# Autodesk Inventor assembly: A2017_T4_06
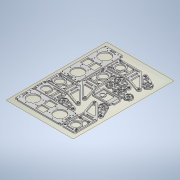
[picture p0: Inventor's stored thumbnail of the model, 180x180]
Saved by Autodesk Inventor 2020 (Build 240168000, 168)
## iProperties
Created: 2021-08-27
Part Number: A2017_T4_06
Document SubType Name: Assembly
Designer: Masato
Author: Masato
## Documents named in this file (10)
- C:\Users\naoki\Documents\Inventor\CitBrains\git_clone\SUSTAINA_ver1_0\AT5_175\SUSTAINA-OP\Cam\A2017_T4_06.iam
- C:\Users\naoki\Documents\Inventor\CitBrains\git_clone\SUSTAINA_ver1_0\AT5_175\SUSTAINA-OP\Cam\DisposableBoard.ipt
- C:\Users\naoki\Documents\Inventor\CitBrains\git_clone\SUSTAINA_ver1_0\AT5_175\SUSTAINA-OP\LowerBody\Ankle\Ankle_side_pitch_frame.ipt
- C:\Users\naoki\Documents\Inventor\CitBrains\git_clone\SUSTAINA_ver1_0\AT5_175\SUSTAINA-OP\UpperBody\Trunk\Trunk_neck_frame.ipt
- C:\Users\naoki\Documents\Inventor\CitBrains\git_clone\SUSTAINA_ver1_0\AT5_175\SUSTAINA-OP\UpperBody\Trunk\Trunk_shoulder_frame.ipt
- C:\Users\naoki\Documents\Inventor\CitBrains\git_clone\SUSTAINA_ver1_0\AT5_175\SUSTAINA-OP\UpperBody\Trunk\Trunk_shoulder_frame_MIR.ipt
- C:\Users\naoki\Documents\Inventor\CitBrains\git_clone\SUSTAINA_ver1_0\AT5_175\SUSTAINA-OP\UpperBody\Trunk\Trunk_waisit_frame.ipt
- C:\Users\naoki\Documents\Inventor\CitBrains\git_clone\SUSTAINA_ver1_0\AT5_175\SUSTAINA-OP\UpperBody\Trunk\Trunk_servo_bottom_frame.ipt
- C:\Users\naoki\Documents\Inventor\CitBrains\git_clone\SUSTAINA_ver1_0\AT4_173\SUSTAINA-OP\UpperBody\Trunk\Trunk_shoulder_frame.ipt
- C:\Users\naoki\Documents\Inventor\CitBrains\git_clone\SUSTAINA_ver1_0\AT4_173\SUSTAINA-OP\UpperBody\Trunk\Trunk_shoulder_frame_MIR.ipt
## Components (15 placed, 7 different names)
1. DisposableBoard:1 — メイト:2, メイト:1, フラッシュ:1, フラッシュ:2, フラッシュ:3, フラッシュ:5, メイト:27, メイト:28, メイト:29, メイト:37, メイト:38, フラッシュ:8, メイト:43, メイト:44, 角度:1, 正接:6, 正接:9
2. Trunk_neck_frame:1 — メイト:6, フラッシュ:6, フラッシュ:7, メイト:16, メイト:17, 正接:2
3. Trunk_shoulder_frame:1 — メイト:9, フラッシュ:4, メイト:15, メイト:45, 正接:3
4. Trunk_shoulder_frame_MIR:1 — メイト:10, フラッシュ:7, メイト:17, メイト:42, メイト:46
5. Trunk_waisit_frame:1 — フラッシュ:3, フラッシュ:4, フラッシュ:5, フラッシュ:6, メイト:15, メイト:16, メイト:19
6. Ankle_side_pitch_frame:2 — メイト:5, メイト:19, 正接:2
7. Ankle_side_pitch_frame:1 — メイト:4, メイト:45, 正接:3, 正接:4
8. Trunk_servo_bottom_frame:2 — メイト:14, 正接:4, メイト:48, 角度:1, メイト:49
9. Trunk_waisit_frame:2 — メイト:27, メイト:42, フラッシュ:8, メイト:47, メイト:52
10. Ankle_side_pitch_frame:6 — メイト:29, メイト:53, 正接:9
11. Ankle_side_pitch_frame:7 — メイト:28, メイト:51, 正接:7, 正接:8
12. Ankle_side_pitch_frame:8 — メイト:37, メイト:50, 正接:5, メイト:51
13. Ankle_side_pitch_frame:9 — メイト:38, メイト:49, メイト:50, 正接:6
14. Trunk_shoulder_frame:2 — メイト:44, メイト:46, メイト:47, メイト:48, 正接:5, 正接:7
15. Trunk_shoulder_frame_MIR:2 — メイト:43, 正接:8, メイト:52, メイト:53
## Relationships (46: Mate 29, Flush 8, Tangent 8, Angle 1)
- メイト:2 [Mate]: DisposableBoard:1
- メイト:1 [Mate]: DisposableBoard:1
- フラッシュ:1 [Flush]: DisposableBoard:1
- フラッシュ:2 [Flush]: DisposableBoard:1
- メイト:4 [Mate]: Ankle_side_pitch_frame:1
- メイト:5 [Mate]: Ankle_side_pitch_frame:2
- メイト:6 [Mate]: Trunk_neck_frame:1
- メイト:9 [Mate]: Trunk_shoulder_frame:1
- メイト:10 [Mate]: Trunk_shoulder_frame_MIR:1
- メイト:14 [Mate]: Trunk_servo_bottom_frame:2
- フラッシュ:3 [Flush] (2 mm): DisposableBoard:1 ↔ Trunk_waisit_frame:1
- フラッシュ:4 [Flush]: Trunk_shoulder_frame:1 ↔ Trunk_waisit_frame:1
- フラッシュ:5 [Flush] (2 mm): DisposableBoard:1 ↔ Trunk_waisit_frame:1
- フラッシュ:6 [Flush]: Trunk_neck_frame:1 ↔ Trunk_waisit_frame:1
- フラッシュ:7 [Flush]: Trunk_neck_frame:1 ↔ Trunk_shoulder_frame_MIR:1
- メイト:15 [Mate] (2.5 mm): Trunk_shoulder_frame:1 ↔ Trunk_waisit_frame:1
- メイト:16 [Mate] (2.5 mm): Trunk_neck_frame:1 ↔ Trunk_waisit_frame:1
- メイト:17 [Mate] (2.5 mm): Trunk_neck_frame:1 ↔ Trunk_shoulder_frame_MIR:1
- メイト:19 [Mate] (2.5 mm): Trunk_waisit_frame:1 ↔ Ankle_side_pitch_frame:2
- 正接:2 [Tangent] (2.5 mm): Trunk_neck_frame:1 ↔ Ankle_side_pitch_frame:2
- メイト:27 [Mate]: DisposableBoard:1 ↔ Trunk_waisit_frame:2
- メイト:28 [Mate]: DisposableBoard:1 ↔ Ankle_side_pitch_frame:7
- メイト:29 [Mate]: DisposableBoard:1 ↔ Ankle_side_pitch_frame:6
- メイト:37 [Mate]: DisposableBoard:1 ↔ Ankle_side_pitch_frame:8
- メイト:38 [Mate]: DisposableBoard:1 ↔ Ankle_side_pitch_frame:9
- メイト:42 [Mate] (2.5 mm): Trunk_shoulder_frame_MIR:1 ↔ Trunk_waisit_frame:2
- フラッシュ:8 [Flush] (2.5 mm): DisposableBoard:1 ↔ Trunk_waisit_frame:2
- メイト:43 [Mate]: DisposableBoard:1 ↔ Trunk_shoulder_frame_MIR:2
- メイト:44 [Mate]: DisposableBoard:1 ↔ Trunk_shoulder_frame:2
- メイト:45 [Mate] (2.5 mm): Trunk_shoulder_frame:1 ↔ Ankle_side_pitch_frame:1
- 正接:3 [Tangent]: Trunk_shoulder_frame:1 ↔ Ankle_side_pitch_frame:1
- メイト:46 [Mate] (2.5 mm): Trunk_shoulder_frame_MIR:1 ↔ Trunk_shoulder_frame:2
- メイト:47 [Mate] (2.5 mm): Trunk_waisit_frame:2 ↔ Trunk_shoulder_frame:2
- 正接:4 [Tangent] (2.5 mm): Ankle_side_pitch_frame:1 ↔ Trunk_servo_bottom_frame:2
- メイト:48 [Mate] (2.5 mm): Trunk_servo_bottom_frame:2 ↔ Trunk_shoulder_frame:2
- 角度:1 [Angle] (0 deg): DisposableBoard:1 ↔ Trunk_servo_bottom_frame:2
- メイト:49 [Mate] (2.5 mm): Trunk_servo_bottom_frame:2 ↔ Ankle_side_pitch_frame:9
- メイト:50 [Mate] (2.5 mm): Ankle_side_pitch_frame:8 ↔ Ankle_side_pitch_frame:9
- 正接:5 [Tangent] (2.5 mm): Ankle_side_pitch_frame:8 ↔ Trunk_shoulder_frame:2
- 正接:6 [Tangent] (3 mm): DisposableBoard:1 ↔ Ankle_side_pitch_frame:9
- メイト:51 [Mate] (2.5 mm): Ankle_side_pitch_frame:7 ↔ Ankle_side_pitch_frame:8
- 正接:7 [Tangent] (2.5 mm): Ankle_side_pitch_frame:7 ↔ Trunk_shoulder_frame:2
- 正接:8 [Tangent] (2.5 mm): Ankle_side_pitch_frame:7 ↔ Trunk_shoulder_frame_MIR:2
- メイト:52 [Mate] (2.5 mm): Trunk_waisit_frame:2 ↔ Trunk_shoulder_frame_MIR:2
- メイト:53 [Mate] (2.5 mm): Ankle_side_pitch_frame:6 ↔ Trunk_shoulder_frame_MIR:2
- 正接:9 [Tangent] (3 mm): DisposableBoard:1 ↔ Ankle_side_pitch_frame:6
